# Autodesk Inventor assembly: Elektro_asm
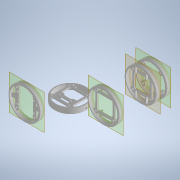
[picture p0: Inventor's stored thumbnail of the model, 180x180]
Saved by Autodesk Inventor 2020 (Build 240168000, 168)
## iProperties
Created: 2022-03-10
Part Number: Elektro_asm
Document SubType Name: Assembly
Designer: sp
Author: sp
## Documents named in this file (5)
- C:\Users\sp\Documents\Rocket\rocket\CAD\Elektro_asm.iam
- C:\Users\sp\Documents\Rocket\rocket\CAD\Electro_unit.ipt
- C:\Users\sp\Documents\Rocket\rocket\CAD\Elektro_Gyro.ipt
- C:\Users\sp\Documents\Rocket\rocket\CAD\Electro_gps.ipt
- C:\Users\sp\Documents\Rocket\rocket\CAD\Electro_bat_down.ipt
## Components (5 placed, 4 different names)
1. Electro_unit:1 — Einfügen:1
2. Elektro_Gyro:1
3. Electro_gps:1
4. Electro_bat_down:1 — Einfügen:2
5. Electro_bat_down:2 — Einfügen:1, Einfügen:2
## Relationships (2: Insert 2)
- Einfügen:1 [Insert] (10 mm): Electro_unit:1 ↔ Electro_bat_down:2
- Einfügen:2 [Insert] (60 mm): Electro_bat_down:1 ↔ Electro_bat_down:2
